# Autodesk Inventor assembly: Final E core
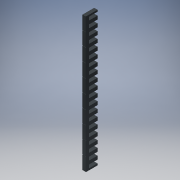
[picture p0: Inventor's stored thumbnail of the model, 180x180]
Saved by Autodesk Inventor 2019 (Build 230136000, 136)
## iProperties
Created: 2021-07-12
Part Number: Final E core
Document SubType Name: Assembly
Designer: pensun
Author: pensun
## Documents named in this file (2)
- C:\Pengpeng\02 coreWithCoil(Ecore)\Hyperloop\Track\Final E core.iam
- C:\Pengpeng\02 coreWithCoil(Ecore)\Hyperloop\E core\Ecorewithoutcoil.ipt
## Components (10 placed, 1 different names)
1. Ecorewithoutcoil:1
2. Ecorewithoutcoil:2
3. Ecorewithoutcoil:3
4. Ecorewithoutcoil:4
5. Ecorewithoutcoil:5
6. Ecorewithoutcoil:6
7. Ecorewithoutcoil:7
8. Ecorewithoutcoil:8
9. Ecorewithoutcoil:9
10. Ecorewithoutcoil:10
## Component patterns: (10 elements, first: Ecorewithoutcoil:1)
